# Autodesk Inventor assembly: PUERTA SP40-02 INT-EXT 2073x761
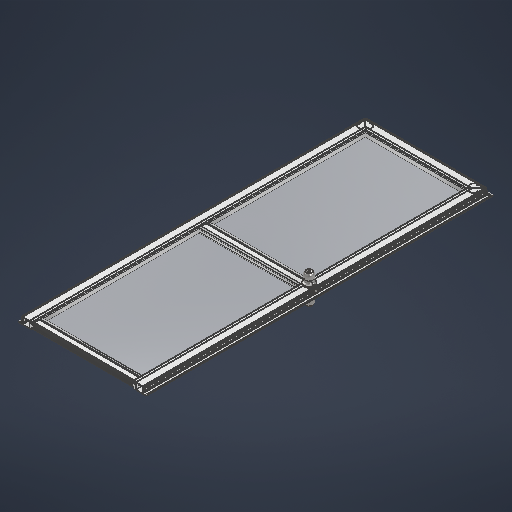
[picture p0: Inventor's stored thumbnail of the model, 512x512]
Saved by Autodesk Inventor 2025 (Build 290162000, 162)
## iProperties
Created: 2026-02-13
Part Number: PUERTA SP40-02 INT-EXT 2073x761
Document SubType Name: Assembly
Designer: ROLANDO
Author: ROLANDO
## Documents named in this file (31)
- C:\Users\rolan\OneDrive\Documentos\Inventor\Projects\CARPINTERIA ALUMINIO\PUERTAS Y VENTANAS\PUERTAS\PUERTAS\ENSAMBLES\PUERTA SP40-02 INT 2100x800 Doble cristal.iam
- C:\Users\rolan\OneDrive\Documentos\Inventor\Projects\CARPINTERIA ALUMINIO\PUERTAS Y VENTANAS\PUERTAS\PUERTAS\PIEZAS\PUERTA SP40-02 INT 2100x800 Doble cristal\SP40-02 HOJA PUERTA BATIENTE INT - EXT 761 mm.ipt
- SP40-02 HOJA PUERTA BATIENTE INT - EXT 761 mm.ipt
- C:\Users\rolan\OneDrive\Documentos\Inventor\Projects\CARPINTERIA ALUMINIO\PUERTAS Y VENTANAS\PUERTAS\PUERTAS\PIEZAS\PUERTA SP40-02 INT 2100x800 Doble cristal\SP40-02 HOJA PUERTA BATIENTE INT - EXT 2073 mm.ipt
- SP40-02 HOJA PUERTA BATIENTE INT - EXT 2073 mm.ipt
- C:\Users\rolan\OneDrive\Documentos\Inventor\Projects\CARPINTERIA ALUMINIO\PUERTAS Y VENTANAS\PUERTAS\PUERTAS\PIEZAS\PUERTA SP40-02 INT 2100x800 Doble cristal\BRA-15 ESCUADRA UNIÓN 45 GRUESA 37 mm.ipt
- C:\Users\rolan\OneDrive\Documentos\Inventor\Projects\CARPINTERIA ALUMINIO\PUERTAS Y VENTANAS\PUERTAS\PUERTAS\PIEZAS\PUERTA SP40-02 INT 2100x800 Doble cristal\JUNTA EXT DE PERFILES CURVA 2073 mm.ipt
- JUNTA EXT DE PERFILES CURVA 2073 mm.ipt
- C:\Users\rolan\OneDrive\Documentos\Inventor\Projects\CARPINTERIA ALUMINIO\PUERTAS Y VENTANAS\PUERTAS\PUERTAS\PIEZAS\PUERTA SP40-02 INT 2100x800 Doble cristal\JUNTA EXT DE PERFILES CURVA 761 mm.ipt
- JUNTA EXT DE PERFILES CURVA 761 mm.ipt
- C:\Users\rolan\OneDrive\Documentos\Inventor\Projects\CARPINTERIA ALUMINIO\PUERTAS Y VENTANAS\PUERTAS\PUERTAS\PIEZAS\PUERTA SP40-02 INT 2100x800 Doble cristal\JUNTA INT DE PERFILES RECTA 2073 mm.ipt
- JUNTA INT DE PERFILES RECTA 2073 mm.ipt
- C:\Users\rolan\OneDrive\Documentos\Inventor\Projects\CARPINTERIA ALUMINIO\PUERTAS Y VENTANAS\PUERTAS\PUERTAS\PIEZAS\PUERTA SP40-02 INT 2100x800 Doble cristal\JUNTA INT DE PERFILES RECTA 761 mm.ipt
- JUNTA INT DE PERFILES RECTA 761 mm.ipt
- C:\Users\rolan\OneDrive\Documentos\Inventor\Projects\CARPINTERIA ALUMINIO\PUERTAS Y VENTANAS\PUERTAS\PUERTAS\PIEZAS\PUERTA SP40-02 INT 2100x800 Doble cristal\SP40-02 HOJA PUERTA BATIENTE INT - EXT 2073 mm_MIR.ipt
- C:\Users\rolan\OneDrive\Documentos\Inventor\Projects\CARPINTERIA ALUMINIO\PUERTAS Y VENTANAS\PUERTAS\PUERTAS\PIEZAS\PUERTA SP40-02 INT 2100x800 Doble cristal\JUNTA EXT DE PERFILES CURVA 2073 mm_MIR.ipt
- C:\Users\rolan\OneDrive\Documentos\Inventor\Projects\CARPINTERIA ALUMINIO\PUERTAS Y VENTANAS\PUERTAS\PUERTAS\PIEZAS\PUERTA SP40-02 INT 2100x800 Doble cristal\JUNTA INT DE PERFILES RECTA 2073 mm_MIR.ipt
- C:\Users\rolan\OneDrive\Documentos\Inventor\Projects\CARPINTERIA ALUMINIO\PUERTAS Y VENTANAS\PUERTAS\PUERTAS\PIEZAS\PUERTA SP40-02 INT 2100x800 Doble cristal\BRA-15 ESCUADRA UNIÓN 45 GRUESA 37 mm_MIR.ipt
- C:\Users\rolan\OneDrive\Documentos\Inventor\Projects\CARPINTERIA ALUMINIO\PUERTAS Y VENTANAS\PUERTAS\PUERTAS\PIEZAS\PUERTA SP40-02 INT 2100x800 Doble cristal\SP40-04A TRAVESAÑO CENTRAL ZOCALO 602x60.ipt
- C:\Users\rolan\OneDrive\Documentos\Inventor\Projects\CARPINTERIA ALUMINIO\PUERTAS Y VENTANAS\PUERTAS\PUERTAS\PIEZAS\PUERTA SP40-02 INT 2100x800 Doble cristal\JUNTA EXT DE PERFILES RECTA 602 mm ZOCALO.ipt
- JUNTA EXT DE PERFILES RECTA 602 mm ZOCALO.ipt
- C:\Users\rolan\OneDrive\Documentos\Inventor\Projects\CARPINTERIA ALUMINIO\PUERTAS Y VENTANAS\PUERTAS\PUERTAS\PIEZAS\PUERTA SP40-02 INT 2100x800 Doble cristal\PLANCHA DE CRISTAL TRANSPARENTE 953x625 mm.ipt
- C:\Users\rolan\OneDrive\Documentos\Inventor\Projects\CARPINTERIA ALUMINIO\PUERTAS Y VENTANAS\PUERTAS\PUERTAS\PIEZAS\PUERTA SP40-02 INT 2100x800 Doble cristal\JUNTA CRISTAL INT CURVA 2073 mm.ipt
- C:\Users\rolan\OneDrive\Documentos\Inventor\Projects\CARPINTERIA ALUMINIO\PUERTAS Y VENTANAS\PUERTAS\PUERTAS\PIEZAS\PUERTA SP40-02 INT 2100x800 Doble cristal\LOK-58 CERRADURA PICAPORTE (INT).ipt
- C:\Users\rolan\OneDrive\Documentos\Inventor\Projects\CARPINTERIA ALUMINIO\PUERTAS Y VENTANAS\PUERTAS\PUERTAS\PIEZAS\PUERTA SP40-02 INT 2100x800 Doble cristal\JUNTA CRISTAL INT CURVA 2073 mm_MIR.ipt
- C:\Users\rolan\OneDrive\Documentos\Inventor\Projects\CARPINTERIA ALUMINIO\PUERTAS Y VENTANAS\PUERTAS\PUERTAS\PIEZAS\PUERTA SP40-02 INT 2100x800 Doble cristal\JUNTA CRISTAL INT CURVA 761 mm.ipt
- C:\Users\rolan\OneDrive\Documentos\Inventor\Projects\CARPINTERIA ALUMINIO\PUERTAS Y VENTANAS\ACCESORIOS\BISAGRAS\ENSAMBLES\HIN-61 BISAGRA (P2 PUERTA).iam
- C:\Users\rolan\OneDrive\Documentos\Inventor\Projects\CARPINTERIA ALUMINIO\PUERTAS Y VENTANAS\ACCESORIOS\CERRADURAS\LOK-58 CERRADURA PICAPORTE\LOK-58 CERRADURA PICAPORTE (PASADOR).ipt
- C:\Users\rolan\OneDrive\Documentos\Inventor\Projects\CARPINTERIA ALUMINIO\PUERTAS Y VENTANAS\ACCESORIOS\CERRADURAS\LOK-58 CERRADURA PICAPORTE\LOK-58 CERRADURA PICAPORTE (EXT).ipt
- C:\Users\rolan\Documents\Inventor\Content Center Files\R2025\es-ES\AS 1420\AS 1420 - 1973 - M4 x 30.ipt
- C:\Users\rolan\OneDrive\Documentos\Inventor\Projects\CARPINTERIA ALUMINIO\PUERTAS Y VENTANAS\PUERTAS\PUERTAS\PIEZAS\PUERTA SP40-02 INT 2100x800 Doble cristal\JUNTA CRISTAL INT RECTA 602 mm ZOCALO.ipt
## Components (38 placed, 23 different names)
1. SP40-02 HOJA PUERTA BATIENTE INT - EXT 761 mm:1 — Coincidencia:1, Coincidencia:3, Coincidencia:4, Coincidencia:5, Coincidencia:13, Coincidencia:14, Nivelación:5, Coincidencia:15, Coincidencia:16, Nivelación:6, Nivelación:9, Coincidencia:23, Coincidencia:25, Coincidencia:26, Coincidencia:29, Coincidencia:37, Coincidencia:38, Coincidencia:48, Nivelación:20, Coincidencia:49, Nivelación:21
2. SP40-02 HOJA PUERTA BATIENTE INT - EXT 2073 mm:1 — Coincidencia:2, Coincidencia:4, Coincidencia:5, Coincidencia:6, Coincidencia:7, Coincidencia:8, Nivelación:2, Coincidencia:11, Coincidencia:12, Nivelación:4, Coincidencia:36, Coincidencia:43, Coincidencia:44, Nivelación:16, Coincidencia:50, Coincidencia:51, Coincidencia:52, Coincidencia:53, Nivelación:22, Insertar:1, Insertar:2, Insertar:3, Insertar:4
3. BRA-15 ESCUADRA UNIÓN 45 GRUESA 37 mm:1 — Coincidencia:1, Coincidencia:2, Coincidencia:3, Coincidencia:6
4. JUNTA EXT DE PERFILES CURVA 761 mm:1 — Coincidencia:15, Coincidencia:16, Nivelación:6
5. JUNTA EXT DE PERFILES CURVA 2073 mm:1 — Coincidencia:7, Coincidencia:8, Nivelación:2
6. JUNTA INT DE PERFILES RECTA 761 mm:1 — Coincidencia:13, Coincidencia:14, Nivelación:5
7. JUNTA INT DE PERFILES RECTA 2073 mm:1 — Coincidencia:11, Coincidencia:12, Nivelación:4
8. JUNTA CRISTAL INT CURVA 761 mm:1 — Coincidencia:48, Nivelación:20, Coincidencia:49
9. JUNTA CRISTAL INT CURVA 2073 mm:1 — Coincidencia:43, Coincidencia:44, Nivelación:16
10. SP40-02 HOJA PUERTA BATIENTE INT - EXT 2073 mm_MIR:1 — Coincidencia:18, Nivelación:7, Coincidencia:19, Coincidencia:20, Nivelación:8, Coincidencia:21, Coincidencia:22, Coincidencia:24, Coincidencia:25, Coincidencia:26, Coincidencia:27, Nivelación:10, Coincidencia:28, Nivelación:11, Nivelación:12, Coincidencia:41, Nivelación:17, Nivelación:18, Nivelación:19, Coincidencia:46, Coincidencia:47, Coincidencia:54, Coincidencia:55, Coincidencia:56, Coincidencia:57, Coincidencia:58, Coincidencia:59, Coincidencia:60, Coincidencia:61, Coincidencia:62, Insertar:5, Insertar:6, Insertar:7, Insertar:8
11. BRA-15 ESCUADRA UNIÓN 45 GRUESA 37 mm_MIR:1 — Nivelación:9, Coincidencia:18, Coincidencia:23, Coincidencia:24
12. JUNTA EXT DE PERFILES CURVA 2073 mm_MIR:1 — Nivelación:7, Coincidencia:19, Coincidencia:20
13. JUNTA INT DE PERFILES RECTA 2073 mm_MIR:1 — Nivelación:8, Coincidencia:21, Coincidencia:22
14. SP40-04A TRAVESAÑO CENTRAL ZOCALO 602x60:1 — Coincidencia:28, Nivelación:11, Nivelación:12, Coincidencia:30, Coincidencia:31, Nivelación:13, Coincidencia:63, Coincidencia:64, Nivelación:23
15. SP40-04A TRAVESAÑO CENTRAL ZOCALO 602x60:2 — Coincidencia:27, Nivelación:10, Coincidencia:29, Coincidencia:32, Coincidencia:33, Nivelación:14, Coincidencia:34, Coincidencia:35, Nivelación:15, Coincidencia:39, Coincidencia:40, Coincidencia:65, Coincidencia:66, Nivelación:24, Coincidencia:67, Coincidencia:68, Nivelación:25
16. JUNTA EXT DE PERFILES RECTA 602 mm ZOCALO:1 — Coincidencia:32, Coincidencia:33, Nivelación:14
17. JUNTA EXT DE PERFILES RECTA 602 mm ZOCALO:2 — Coincidencia:34, Coincidencia:35, Nivelación:15
18. JUNTA EXT DE PERFILES RECTA 602 mm ZOCALO:3 — Coincidencia:30, Coincidencia:31, Nivelación:13
19. JUNTA CRISTAL INT CURVA 2073 mm_MIR:1 — Nivelación:18, Nivelación:19, Coincidencia:46, Coincidencia:47
20. JUNTA CRISTAL INT RECTA 602 mm ZOCALO:1 — Coincidencia:65, Coincidencia:66, Nivelación:24
21. JUNTA CRISTAL INT RECTA 602 mm ZOCALO:2 — Coincidencia:67, Coincidencia:68, Nivelación:25
22. JUNTA CRISTAL INT RECTA 602 mm ZOCALO:3 — Coincidencia:63, Coincidencia:64, Nivelación:23
23. PLANCHA DE CRISTAL TRANSPARENTE 953x625 mm:1 — Coincidencia:36, Coincidencia:37, Coincidencia:38
24. PLANCHA DE CRISTAL TRANSPARENTE 953x625 mm:2 — Coincidencia:39, Coincidencia:40, Coincidencia:41
25. LOK-58 CERRADURA PICAPORTE (EXT):1 — Coincidencia:60, Coincidencia:61, Coincidencia:62
26. LOK-58 CERRADURA PICAPORTE (INT):1 — Coincidencia:57, Coincidencia:58, Coincidencia:59
27. LOK-58 CERRADURA PICAPORTE (PASADOR):1 — Coincidencia:54, Coincidencia:55, Coincidencia:56
28. HIN-61 BISAGRA (P2 PUERTA):3 [sub-assembly] — Coincidencia:52, Coincidencia:53, Nivelación:22
29. AS 1420 - Métrico M4 x 30:1 — Insertar:1
30. AS 1420 - Métrico M4 x 30:2 — Insertar:2
31. AS 1420 - Métrico M4 x 30:3 — Insertar:3
32. AS 1420 - Métrico M4 x 30:4 — Insertar:4
33. AS 1420 - Métrico M4 x 30:5 — Insertar:5
34. AS 1420 - Métrico M4 x 30:6 — Insertar:6
35. AS 1420 - Métrico M4 x 30:7 — Insertar:7
36. AS 1420 - Métrico M4 x 30:8 — Insertar:8
37. HIN-61 BISAGRA (P2 PUERTA):1 [sub-assembly] — Coincidencia:50, Coincidencia:51, Nivelación:21
38. HIN-61 BISAGRA (P2 PUERTA):2 [sub-assembly]
## Component patterns: (2 elements, first: HIN-61 BISAGRA (P2 PUERTA):1)
## Relationships (94: Mate 63, Flush 23, Insert 8)
- Coincidencia:1 [Mate]: SP40-02 HOJA PUERTA BATIENTE INT - EXT 761 mm:1 ↔ BRA-15 ESCUADRA UNIÓN 45 GRUESA 37 mm:1
- Coincidencia:2 [Mate]: SP40-02 HOJA PUERTA BATIENTE INT - EXT 2073 mm:1 ↔ BRA-15 ESCUADRA UNIÓN 45 GRUESA 37 mm:1
- Coincidencia:3 [Mate] (0.2 mm): SP40-02 HOJA PUERTA BATIENTE INT - EXT 761 mm:1 ↔ BRA-15 ESCUADRA UNIÓN 45 GRUESA 37 mm:1
- Coincidencia:4 [Mate]: SP40-02 HOJA PUERTA BATIENTE INT - EXT 761 mm:1 ↔ SP40-02 HOJA PUERTA BATIENTE INT - EXT 2073 mm:1
- Coincidencia:5 [Mate]: SP40-02 HOJA PUERTA BATIENTE INT - EXT 761 mm:1 ↔ SP40-02 HOJA PUERTA BATIENTE INT - EXT 2073 mm:1
- Coincidencia:6 [Mate] (0.1 mm): SP40-02 HOJA PUERTA BATIENTE INT - EXT 2073 mm:1 ↔ BRA-15 ESCUADRA UNIÓN 45 GRUESA 37 mm:1
- Coincidencia:7 [Mate]: SP40-02 HOJA PUERTA BATIENTE INT - EXT 2073 mm:1 ↔ JUNTA EXT DE PERFILES CURVA 2073 mm:1
- Coincidencia:8 [Mate]: SP40-02 HOJA PUERTA BATIENTE INT - EXT 2073 mm:1 ↔ JUNTA EXT DE PERFILES CURVA 2073 mm:1
- Nivelación:2 [Flush]: SP40-02 HOJA PUERTA BATIENTE INT - EXT 2073 mm:1 ↔ JUNTA EXT DE PERFILES CURVA 2073 mm:1
- Coincidencia:11 [Mate]: SP40-02 HOJA PUERTA BATIENTE INT - EXT 2073 mm:1 ↔ JUNTA INT DE PERFILES RECTA 2073 mm:1
- Coincidencia:12 [Mate]: SP40-02 HOJA PUERTA BATIENTE INT - EXT 2073 mm:1 ↔ JUNTA INT DE PERFILES RECTA 2073 mm:1
- Nivelación:4 [Flush]: SP40-02 HOJA PUERTA BATIENTE INT - EXT 2073 mm:1 ↔ JUNTA INT DE PERFILES RECTA 2073 mm:1
- Coincidencia:13 [Mate]: SP40-02 HOJA PUERTA BATIENTE INT - EXT 761 mm:1 ↔ JUNTA INT DE PERFILES RECTA 761 mm:1
- Coincidencia:14 [Mate]: SP40-02 HOJA PUERTA BATIENTE INT - EXT 761 mm:1 ↔ JUNTA INT DE PERFILES RECTA 761 mm:1
- Nivelación:5 [Flush]: SP40-02 HOJA PUERTA BATIENTE INT - EXT 761 mm:1 ↔ JUNTA INT DE PERFILES RECTA 761 mm:1
- Coincidencia:15 [Mate]: SP40-02 HOJA PUERTA BATIENTE INT - EXT 761 mm:1 ↔ JUNTA EXT DE PERFILES CURVA 761 mm:1
- Coincidencia:16 [Mate]: SP40-02 HOJA PUERTA BATIENTE INT - EXT 761 mm:1 ↔ JUNTA EXT DE PERFILES CURVA 761 mm:1
- Nivelación:6 [Flush]: SP40-02 HOJA PUERTA BATIENTE INT - EXT 761 mm:1 ↔ JUNTA EXT DE PERFILES CURVA 761 mm:1
- Nivelación:9 [Flush]: SP40-02 HOJA PUERTA BATIENTE INT - EXT 761 mm:1 ↔ BRA-15 ESCUADRA UNIÓN 45 GRUESA 37 mm_MIR:1
- Coincidencia:18 [Mate]: SP40-02 HOJA PUERTA BATIENTE INT - EXT 2073 mm_MIR:1 ↔ BRA-15 ESCUADRA UNIÓN 45 GRUESA 37 mm_MIR:1
- Nivelación:7 [Flush]: SP40-02 HOJA PUERTA BATIENTE INT - EXT 2073 mm_MIR:1 ↔ JUNTA EXT DE PERFILES CURVA 2073 mm_MIR:1
- Coincidencia:19 [Mate]: SP40-02 HOJA PUERTA BATIENTE INT - EXT 2073 mm_MIR:1 ↔ JUNTA EXT DE PERFILES CURVA 2073 mm_MIR:1
- Coincidencia:20 [Mate]: SP40-02 HOJA PUERTA BATIENTE INT - EXT 2073 mm_MIR:1 ↔ JUNTA EXT DE PERFILES CURVA 2073 mm_MIR:1
- Nivelación:8 [Flush]: SP40-02 HOJA PUERTA BATIENTE INT - EXT 2073 mm_MIR:1 ↔ JUNTA INT DE PERFILES RECTA 2073 mm_MIR:1
- Coincidencia:21 [Mate]: SP40-02 HOJA PUERTA BATIENTE INT - EXT 2073 mm_MIR:1 ↔ JUNTA INT DE PERFILES RECTA 2073 mm_MIR:1
- Coincidencia:22 [Mate]: SP40-02 HOJA PUERTA BATIENTE INT - EXT 2073 mm_MIR:1 ↔ JUNTA INT DE PERFILES RECTA 2073 mm_MIR:1
- Coincidencia:23 [Mate] (0.2 mm): SP40-02 HOJA PUERTA BATIENTE INT - EXT 761 mm:1 ↔ BRA-15 ESCUADRA UNIÓN 45 GRUESA 37 mm_MIR:1
- Coincidencia:24 [Mate] (0.1 mm): SP40-02 HOJA PUERTA BATIENTE INT - EXT 2073 mm_MIR:1 ↔ BRA-15 ESCUADRA UNIÓN 45 GRUESA 37 mm_MIR:1
- Coincidencia:25 [Mate]: SP40-02 HOJA PUERTA BATIENTE INT - EXT 761 mm:1 ↔ SP40-02 HOJA PUERTA BATIENTE INT - EXT 2073 mm_MIR:1
- Coincidencia:26 [Mate]: SP40-02 HOJA PUERTA BATIENTE INT - EXT 761 mm:1 ↔ SP40-02 HOJA PUERTA BATIENTE INT - EXT 2073 mm_MIR:1
- Coincidencia:27 [Mate]: SP40-02 HOJA PUERTA BATIENTE INT - EXT 2073 mm_MIR:1 ↔ SP40-04A TRAVESAÑO CENTRAL ZOCALO 602x60:2
- Nivelación:10 [Flush]: SP40-02 HOJA PUERTA BATIENTE INT - EXT 2073 mm_MIR:1 ↔ SP40-04A TRAVESAÑO CENTRAL ZOCALO 602x60:2
- Coincidencia:28 [Mate]: SP40-02 HOJA PUERTA BATIENTE INT - EXT 2073 mm_MIR:1 ↔ SP40-04A TRAVESAÑO CENTRAL ZOCALO 602x60:1
- Nivelación:11 [Flush]: SP40-02 HOJA PUERTA BATIENTE INT - EXT 2073 mm_MIR:1 ↔ SP40-04A TRAVESAÑO CENTRAL ZOCALO 602x60:1
- Nivelación:12 [Flush]: SP40-02 HOJA PUERTA BATIENTE INT - EXT 2073 mm_MIR:1 ↔ SP40-04A TRAVESAÑO CENTRAL ZOCALO 602x60:1
- Coincidencia:29 [Mate] (930.25 mm): SP40-02 HOJA PUERTA BATIENTE INT - EXT 761 mm:1 ↔ SP40-04A TRAVESAÑO CENTRAL ZOCALO 602x60:2
- Coincidencia:30 [Mate]: SP40-04A TRAVESAÑO CENTRAL ZOCALO 602x60:1 ↔ JUNTA EXT DE PERFILES RECTA 602 mm ZOCALO:3
- Coincidencia:31 [Mate]: SP40-04A TRAVESAÑO CENTRAL ZOCALO 602x60:1 ↔ JUNTA EXT DE PERFILES RECTA 602 mm ZOCALO:3
- Nivelación:13 [Flush]: SP40-04A TRAVESAÑO CENTRAL ZOCALO 602x60:1 ↔ JUNTA EXT DE PERFILES RECTA 602 mm ZOCALO:3
- Coincidencia:32 [Mate]: SP40-04A TRAVESAÑO CENTRAL ZOCALO 602x60:2 ↔ JUNTA EXT DE PERFILES RECTA 602 mm ZOCALO:1
- Coincidencia:33 [Mate]: SP40-04A TRAVESAÑO CENTRAL ZOCALO 602x60:2 ↔ JUNTA EXT DE PERFILES RECTA 602 mm ZOCALO:1
- Nivelación:14 [Flush]: SP40-04A TRAVESAÑO CENTRAL ZOCALO 602x60:2 ↔ JUNTA EXT DE PERFILES RECTA 602 mm ZOCALO:1
- Coincidencia:34 [Mate]: SP40-04A TRAVESAÑO CENTRAL ZOCALO 602x60:2 ↔ JUNTA EXT DE PERFILES RECTA 602 mm ZOCALO:2
- Coincidencia:35 [Mate]: SP40-04A TRAVESAÑO CENTRAL ZOCALO 602x60:2 ↔ JUNTA EXT DE PERFILES RECTA 602 mm ZOCALO:2
- Nivelación:15 [Flush]: SP40-04A TRAVESAÑO CENTRAL ZOCALO 602x60:2 ↔ JUNTA EXT DE PERFILES RECTA 602 mm ZOCALO:2
- Coincidencia:36 [Mate] (2.9 mm): SP40-02 HOJA PUERTA BATIENTE INT - EXT 2073 mm:1 ↔ PLANCHA DE CRISTAL TRANSPARENTE 953x625 mm:1
- Coincidencia:37 [Mate] (2.5 mm): SP40-02 HOJA PUERTA BATIENTE INT - EXT 761 mm:1 ↔ PLANCHA DE CRISTAL TRANSPARENTE 953x625 mm:1
- Coincidencia:38 [Mate] (3.9 mm): SP40-02 HOJA PUERTA BATIENTE INT - EXT 761 mm:1 ↔ PLANCHA DE CRISTAL TRANSPARENTE 953x625 mm:1
- Coincidencia:39 [Mate] (2.5 mm): SP40-04A TRAVESAÑO CENTRAL ZOCALO 602x60:2 ↔ PLANCHA DE CRISTAL TRANSPARENTE 953x625 mm:2
- Coincidencia:40 [Mate] (3.9 mm): SP40-04A TRAVESAÑO CENTRAL ZOCALO 602x60:2 ↔ PLANCHA DE CRISTAL TRANSPARENTE 953x625 mm:2
- Coincidencia:41 [Mate] (2.9 mm): SP40-02 HOJA PUERTA BATIENTE INT - EXT 2073 mm_MIR:1 ↔ PLANCHA DE CRISTAL TRANSPARENTE 953x625 mm:2
- Coincidencia:43 [Mate]: SP40-02 HOJA PUERTA BATIENTE INT - EXT 2073 mm:1 ↔ JUNTA CRISTAL INT CURVA 2073 mm:1
- Coincidencia:44 [Mate]: SP40-02 HOJA PUERTA BATIENTE INT - EXT 2073 mm:1 ↔ JUNTA CRISTAL INT CURVA 2073 mm:1
- Nivelación:16 [Flush]: SP40-02 HOJA PUERTA BATIENTE INT - EXT 2073 mm:1 ↔ JUNTA CRISTAL INT CURVA 2073 mm:1
- Nivelación:17 [Flush] (-20.15 mm): SP40-02 HOJA PUERTA BATIENTE INT - EXT 2073 mm_MIR:1
- Nivelación:18 [Flush]: SP40-02 HOJA PUERTA BATIENTE INT - EXT 2073 mm_MIR:1 ↔ JUNTA CRISTAL INT CURVA 2073 mm_MIR:1
- Nivelación:19 [Flush]: SP40-02 HOJA PUERTA BATIENTE INT - EXT 2073 mm_MIR:1 ↔ JUNTA CRISTAL INT CURVA 2073 mm_MIR:1
- Coincidencia:46 [Mate]: SP40-02 HOJA PUERTA BATIENTE INT - EXT 2073 mm_MIR:1 ↔ JUNTA CRISTAL INT CURVA 2073 mm_MIR:1
- Coincidencia:47 [Mate]: SP40-02 HOJA PUERTA BATIENTE INT - EXT 2073 mm_MIR:1 ↔ JUNTA CRISTAL INT CURVA 2073 mm_MIR:1
- Coincidencia:48 [Mate]: SP40-02 HOJA PUERTA BATIENTE INT - EXT 761 mm:1 ↔ JUNTA CRISTAL INT CURVA 761 mm:1
- Nivelación:20 [Flush]: SP40-02 HOJA PUERTA BATIENTE INT - EXT 761 mm:1 ↔ JUNTA CRISTAL INT CURVA 761 mm:1
- Coincidencia:49 [Mate]: SP40-02 HOJA PUERTA BATIENTE INT - EXT 761 mm:1 ↔ JUNTA CRISTAL INT CURVA 761 mm:1
- Coincidencia:50 [Mate]: SP40-02 HOJA PUERTA BATIENTE INT - EXT 2073 mm:1 ↔ HIN-61 BISAGRA (P2 PUERTA):1
- Coincidencia:51 [Mate]: SP40-02 HOJA PUERTA BATIENTE INT - EXT 2073 mm:1 ↔ HIN-61 BISAGRA (P2 PUERTA):1
- Nivelación:21 [Flush] (140 mm): SP40-02 HOJA PUERTA BATIENTE INT - EXT 761 mm:1 ↔ HIN-61 BISAGRA (P2 PUERTA):1
- Coincidencia:52 [Mate]: SP40-02 HOJA PUERTA BATIENTE INT - EXT 2073 mm:1 ↔ HIN-61 BISAGRA (P2 PUERTA):3
- Coincidencia:53 [Mate]: SP40-02 HOJA PUERTA BATIENTE INT - EXT 2073 mm:1 ↔ HIN-61 BISAGRA (P2 PUERTA):3
- Nivelación:22 [Flush] (240 mm): SP40-02 HOJA PUERTA BATIENTE INT - EXT 2073 mm:1 ↔ HIN-61 BISAGRA (P2 PUERTA):3
- Coincidencia:54 [Mate]: SP40-02 HOJA PUERTA BATIENTE INT - EXT 2073 mm_MIR:1 ↔ LOK-58 CERRADURA PICAPORTE (PASADOR):1
- Coincidencia:55 [Mate]: SP40-02 HOJA PUERTA BATIENTE INT - EXT 2073 mm_MIR:1 ↔ LOK-58 CERRADURA PICAPORTE (PASADOR):1
- Coincidencia:56 [Mate] (5.75 mm): SP40-02 HOJA PUERTA BATIENTE INT - EXT 2073 mm_MIR:1 ↔ LOK-58 CERRADURA PICAPORTE (PASADOR):1
- Coincidencia:57 [Mate]: SP40-02 HOJA PUERTA BATIENTE INT - EXT 2073 mm_MIR:1 ↔ LOK-58 CERRADURA PICAPORTE (INT):1
- Coincidencia:58 [Mate]: SP40-02 HOJA PUERTA BATIENTE INT - EXT 2073 mm_MIR:1 ↔ LOK-58 CERRADURA PICAPORTE (INT):1
- Coincidencia:59 [Mate]: SP40-02 HOJA PUERTA BATIENTE INT - EXT 2073 mm_MIR:1 ↔ LOK-58 CERRADURA PICAPORTE (INT):1
- Coincidencia:60 [Mate]: SP40-02 HOJA PUERTA BATIENTE INT - EXT 2073 mm_MIR:1 ↔ LOK-58 CERRADURA PICAPORTE (EXT):1
- Coincidencia:61 [Mate]: SP40-02 HOJA PUERTA BATIENTE INT - EXT 2073 mm_MIR:1 ↔ LOK-58 CERRADURA PICAPORTE (EXT):1
- Coincidencia:62 [Mate]: SP40-02 HOJA PUERTA BATIENTE INT - EXT 2073 mm_MIR:1 ↔ LOK-58 CERRADURA PICAPORTE (EXT):1
- Insertar:1: SP40-02 HOJA PUERTA BATIENTE INT - EXT 2073 mm:1 ↔ AS 1420 - Métrico M4 x 30:1
- Insertar:2: SP40-02 HOJA PUERTA BATIENTE INT - EXT 2073 mm:1 ↔ AS 1420 - Métrico M4 x 30:2
- Insertar:3: SP40-02 HOJA PUERTA BATIENTE INT - EXT 2073 mm:1 ↔ AS 1420 - Métrico M4 x 30:3
- Insertar:4: SP40-02 HOJA PUERTA BATIENTE INT - EXT 2073 mm:1 ↔ AS 1420 - Métrico M4 x 30:4
- Insertar:5: SP40-02 HOJA PUERTA BATIENTE INT - EXT 2073 mm_MIR:1 ↔ AS 1420 - Métrico M4 x 30:5
- Insertar:6: SP40-02 HOJA PUERTA BATIENTE INT - EXT 2073 mm_MIR:1 ↔ AS 1420 - Métrico M4 x 30:6
- Insertar:7: SP40-02 HOJA PUERTA BATIENTE INT - EXT 2073 mm_MIR:1 ↔ AS 1420 - Métrico M4 x 30:7
- Insertar:8: SP40-02 HOJA PUERTA BATIENTE INT - EXT 2073 mm_MIR:1 ↔ AS 1420 - Métrico M4 x 30:8
- Coincidencia:63 [Mate]: SP40-04A TRAVESAÑO CENTRAL ZOCALO 602x60:1 ↔ JUNTA CRISTAL INT RECTA 602 mm ZOCALO:3
- Coincidencia:64 [Mate]: SP40-04A TRAVESAÑO CENTRAL ZOCALO 602x60:1 ↔ JUNTA CRISTAL INT RECTA 602 mm ZOCALO:3
- Nivelación:23 [Flush]: SP40-04A TRAVESAÑO CENTRAL ZOCALO 602x60:1 ↔ JUNTA CRISTAL INT RECTA 602 mm ZOCALO:3
- Coincidencia:65 [Mate]: SP40-04A TRAVESAÑO CENTRAL ZOCALO 602x60:2 ↔ JUNTA CRISTAL INT RECTA 602 mm ZOCALO:1
- Coincidencia:66 [Mate]: SP40-04A TRAVESAÑO CENTRAL ZOCALO 602x60:2 ↔ JUNTA CRISTAL INT RECTA 602 mm ZOCALO:1
- Nivelación:24 [Flush]: SP40-04A TRAVESAÑO CENTRAL ZOCALO 602x60:2 ↔ JUNTA CRISTAL INT RECTA 602 mm ZOCALO:1
- Coincidencia:67 [Mate]: SP40-04A TRAVESAÑO CENTRAL ZOCALO 602x60:2 ↔ JUNTA CRISTAL INT RECTA 602 mm ZOCALO:2
- Coincidencia:68 [Mate]: SP40-04A TRAVESAÑO CENTRAL ZOCALO 602x60:2 ↔ JUNTA CRISTAL INT RECTA 602 mm ZOCALO:2
- Nivelación:25 [Flush]: SP40-04A TRAVESAÑO CENTRAL ZOCALO 602x60:2 ↔ JUNTA CRISTAL INT RECTA 602 mm ZOCALO:2
